# Autodesk Inventor assembly: smietnik2_zlozenie
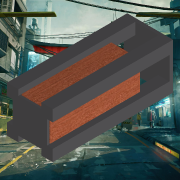
[picture p0: Inventor's stored thumbnail of the model, 180x180]
Saved by Autodesk Inventor 2021 (Build 250183000, 183)
## iProperties
Created: 2025-11-30
Part Number: smietnik2_zlozenie
Document SubType Name: Assembly
Designer: huber
Author: huber
## Documents named in this file (7)
- C:\Users\huber\OneDrive\Pulpit\hackaton BHL\BHL 2025\smietnik2_zlozenie.iam
- C:\Users\huber\OneDrive\Pulpit\hackaton BHL\BHL 2025\smietnik2.ipt
- C:\Users\huber\OneDrive\Pulpit\hackaton BHL\BHL 2025\drewniany obwod.ipt
- C:\Users\huber\OneDrive\Pulpit\hackaton BHL\BHL 2025\drewniany obwod_MIR.ipt
- C:\Users\huber\OneDrive\Pulpit\hackaton BHL\BHL 2025\drewniany obwod_MIR1.ipt
- C:\Users\huber\OneDrive\Pulpit\hackaton BHL\BHL 2025\zlozenie_kompetne_WIZUAL2.iam
- C:\Users\huber\OneDrive\Dokumenty\Inventor\Content Center Files\R2021\en-US\ISO 4016\ISO 4016 - M8 x 40.ipt
## Components (8 placed, 6 different names)
1. smietnik2:1 — Mate:1, Flush:1, Mate:2, Mate:3, Flush:2, Mate:4, Flush:3, Flush:4, Mate:6, Mate:7, Mate:8, Mate:11
2. drewniany obwod:1 — Mate:1, Flush:1, Mate:2
3. drewniany obwod:2 — Mate:3, Flush:2, Mate:4
4. drewniany obwod_MIR:2 — Mate:6, Mate:7, Mate:8, Mate:9, Mate:10
5. drewniany obwod_MIR1:1
6. zlozenie_kompetne_WIZUAL2:1 [sub-assembly] — Mate:9, Mate:10, Mate:11, Insert:1, Insert:2
7. ISO 4016 M8 x 40:1 — Insert:1
8. ISO 4016 M8 x 40:2 — Insert:2
## Relationships (16: Mate 10, Flush 4, Insert 2)
- Mate:1: smietnik2:1 ↔ drewniany obwod:1
- Flush:1: smietnik2:1 ↔ drewniany obwod:1
- Mate:2 (10 mm): smietnik2:1 ↔ drewniany obwod:1
- Mate:3: smietnik2:1 ↔ drewniany obwod:2
- Flush:2: smietnik2:1 ↔ drewniany obwod:2
- Mate:4 (10 mm): smietnik2:1 ↔ drewniany obwod:2
- Flush:3 (-200 mm): smietnik2:1
- Flush:4 (-200 mm): smietnik2:1
- Mate:6: smietnik2:1 ↔ drewniany obwod_MIR:2
- Mate:7: smietnik2:1 ↔ drewniany obwod_MIR:2
- Mate:8 (10 mm): smietnik2:1 ↔ drewniany obwod_MIR:2
- Mate:9: drewniany obwod_MIR:2 ↔ zlozenie_kompetne_WIZUAL2:1
- Mate:10: drewniany obwod_MIR:2 ↔ zlozenie_kompetne_WIZUAL2:1
- Mate:11 (62.5 mm): smietnik2:1 ↔ zlozenie_kompetne_WIZUAL2:1
- Insert:1: zlozenie_kompetne_WIZUAL2:1 ↔ ISO 4016 M8 x 40:1
- Insert:2: zlozenie_kompetne_WIZUAL2:1 ↔ ISO 4016 M8 x 40:2
